# Autodesk Inventor assembly: VexBox
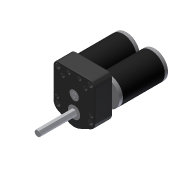
[picture p0: Inventor's stored thumbnail of the model, 180x180]
Saved by Autodesk Inventor 2013 (Build 170138000, 138)
## iProperties
Created: 2012-12-08
Part Number: VexBox
Document SubType Name: Assembly
Designer: Nemo
Mass: 2987.48 g
Surface Area: 2051.7 cm^2
Volume: 949.472 cm^3
Density: 3.14647 g/cm^3
Author: Nemo
## Documents named in this file (15)
- H:\Nemo\Documents\Robotics\VexPro\VexBox\VexBox.iam
- H:\Nemo\Documents\Robotics\VexPro\VexBox\VexBox Casing - Motor Side.ipt
- H:\Nemo\Documents\Robotics\VexPro\VexBox\VexBox Output Shaft.ipt
- H:\Nemo\Documents\Robotics\VexPro\Bearings\Flanged Bearing - 0.5in Round ID x 1.125in OD.ipt
- H:\Nemo\Documents\Robotics\VexPro\Bearings\Flanged Bearing - 0.375in Round ID x 0.875in OD.ipt
- H:\Nemo\Documents\Robotics\VexPro\VexBox\VexBox cluster shaft.ipt
- H:\Nemo\Documents\Robotics\VexPro\VexBox\VexBox Housing - Output Side.ipt
- H:\Nemo\Documents\Robotics\VexPro\Bearings\Flanged Bearing - 0.5in Hex ID x 1.125in OD.ipt
- H:\Nemo\Documents\Robotics\VexPro\Gears\Gear 20dp 10mm key 12T Vex.ipt
- H:\Nemo\Documents\Robotics\VexPro\Gears\Gear 20dp 375hex 14T Vex.ipt
- H:\Nemo\Documents\Robotics\VexPro\Gears\Gear 20dp 375hex 40T Vex.ipt
- H:\Nemo\Documents\Robotics\VexPro\Gears\Gear 20dp 500hex 40T Vex.ipt
- H:\Nemo\Documents\Robotics\COTS Parts\Fasteners\KlipRing for 500hex.ipt
- H:\Nemo\Documents\Robotics\COTS Parts\Motors\CIM motor.ipt
- H:\Nemo\Documents\Robotics\COTS Parts\Fasteners\10-32 SHCS x500.ipt
## Components (20 placed, 14 different names)
1. VexBox Casing - Motor Side:1 — Insert:1, Insert:3, Mate:7, Mate:8, Mate:9, Insert:8, Mate:10, Insert:9, Mate:11, Insert:10, Insert:11, Insert:12, Insert:13
2. VexBox Output Shaft:1 — Insert:2, Mate:1, Insert:7, Angle:2, Rotation:1
3. Flanged Bearing - 0.5in Round ID x 1.125in OD:1 — Insert:1, Insert:2
4. Flanged Bearing - 0.375in Round ID x 0.875in OD:1 — Insert:3, Insert:4, Mate:4
5. VexBox cluster shaft:1 — Insert:4, Mate:2, Angle:1, Mate:5, Angle:3, Rotation:1
6. VexBox Housing - Output Side:1 — Insert:5, Insert:6, Mate:7, Mate:8, Mate:9
7. Flanged Bearing - 0.375in Round ID x 0.875in OD:2 — Insert:5
8. Flanged Bearing - 0.5in Hex ID x 1.125in OD:1 — Insert:6
9. Gear 20dp 10mm key 12T Vex:1 — Mate:12, Angle:4, Mate:13
10. Gear 20dp 375hex 14T Vex:1 — Mate:5, Mate:6, Angle:3
11. Gear 20dp 375hex 40T Vex:1 — Mate:2, Angle:1, Mate:4, Mate:6
12. Gear 20dp 500hex 40T Vex:1 — Mate:1, Angle:2, Mate:3
13. KlipRing for 500hex:1 — Insert:7, Mate:3
14. CIM motor:1 — Insert:9, Mate:11, Mate:12, Angle:4, Mate:13
15. CIM motor:2 — Insert:8, Mate:10, Mate:14, Angle:5, Mate:15
16. Gear 20dp 10mm key 12T Vex:2 — Mate:14, Angle:5, Mate:15
17. 10-32 SHCS x500:1 — Insert:13
18. 10-32 SHCS x500:2 — Insert:12
19. 10-32 SHCS x500:3 — Insert:10
20. 10-32 SHCS x500:4 — Insert:11
## Relationships (34: Mate 15, Insert 13, Angle 5, RelateRotation 1)
- Insert:1: VexBox Casing - Motor Side:1 ↔ Flanged Bearing - 0.5in Round ID x 1.125in OD:1
- Insert:2: VexBox Output Shaft:1 ↔ Flanged Bearing - 0.5in Round ID x 1.125in OD:1
- Insert:3: VexBox Casing - Motor Side:1 ↔ Flanged Bearing - 0.375in Round ID x 0.875in OD:1
- Insert:4: Flanged Bearing - 0.375in Round ID x 0.875in OD:1 ↔ VexBox cluster shaft:1
- Insert:5: VexBox Housing - Output Side:1 ↔ Flanged Bearing - 0.375in Round ID x 0.875in OD:2
- Insert:6: VexBox Housing - Output Side:1 ↔ Flanged Bearing - 0.5in Hex ID x 1.125in OD:1
- Mate:1: VexBox Output Shaft:1 ↔ Gear 20dp 500hex 40T Vex:1
- Insert:7: VexBox Output Shaft:1 ↔ KlipRing for 500hex:1
- Mate:2: VexBox cluster shaft:1 ↔ Gear 20dp 375hex 40T Vex:1
- Angle:1 (0 deg): VexBox cluster shaft:1 ↔ Gear 20dp 375hex 40T Vex:1
- Angle:2 (0 deg): VexBox Output Shaft:1 ↔ Gear 20dp 500hex 40T Vex:1
- Mate:3: Gear 20dp 500hex 40T Vex:1 ↔ KlipRing for 500hex:1
- Mate:4: Flanged Bearing - 0.375in Round ID x 0.875in OD:1 ↔ Gear 20dp 375hex 40T Vex:1
- Mate:5: VexBox cluster shaft:1 ↔ Gear 20dp 375hex 14T Vex:1
- Mate:6: Gear 20dp 375hex 14T Vex:1 ↔ Gear 20dp 375hex 40T Vex:1
- Angle:3 (0 deg): VexBox cluster shaft:1 ↔ Gear 20dp 375hex 14T Vex:1
- Rotation:1 [RelateRotation] (0.35 ul): VexBox Output Shaft:1 ↔ VexBox cluster shaft:1
- Mate:7: VexBox Casing - Motor Side:1 ↔ VexBox Housing - Output Side:1
- Mate:8: VexBox Casing - Motor Side:1 ↔ VexBox Housing - Output Side:1
- Mate:9: VexBox Casing - Motor Side:1 ↔ VexBox Housing - Output Side:1
- Insert:8: VexBox Casing - Motor Side:1 ↔ CIM motor:2
- Mate:10: VexBox Casing - Motor Side:1 ↔ CIM motor:2
- Insert:9: VexBox Casing - Motor Side:1 ↔ CIM motor:1
- Mate:11: VexBox Casing - Motor Side:1 ↔ CIM motor:1
- Mate:12: Gear 20dp 10mm key 12T Vex:1 ↔ CIM motor:1
- Angle:4 (0 deg): Gear 20dp 10mm key 12T Vex:1 ↔ CIM motor:1
- Mate:13 (1.5875 mm): Gear 20dp 10mm key 12T Vex:1 ↔ CIM motor:1
- Mate:14: CIM motor:2 ↔ Gear 20dp 10mm key 12T Vex:2
- Angle:5 (0 deg): CIM motor:2 ↔ Gear 20dp 10mm key 12T Vex:2
- Mate:15 (1.5875 mm): CIM motor:2 ↔ Gear 20dp 10mm key 12T Vex:2
- Insert:10: VexBox Casing - Motor Side:1 ↔ 10-32 SHCS x500:3
- Insert:11: VexBox Casing - Motor Side:1 ↔ 10-32 SHCS x500:4
- Insert:12: VexBox Casing - Motor Side:1 ↔ 10-32 SHCS x500:2
- Insert:13: VexBox Casing - Motor Side:1 ↔ 10-32 SHCS x500:1
